# Autodesk Inventor assembly: hintererAufbau
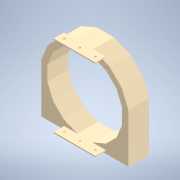
[picture p0: Inventor's stored thumbnail of the model, 180x180]
Saved by Autodesk Inventor 2020.3 (Build 243373010, 373A)
## iProperties
Created: 2021-02-11
Part Number: hintererAufbau
Document SubType Name: Assembly
Designer: Stefan
Author: Stefan
## Documents named in this file (9)
- D:\Stefan\Schule\HTL\Diplomarbeit\git\Inventor\hintererAufbau\hintererAufbau.iam
- D:\Stefan\Schule\HTL\Diplomarbeit\git\Inventor\hintererAufbau\Hauptplatte.ipt
- D:\Stefan\Schule\HTL\Diplomarbeit\git\Inventor\hintererAufbau\InnenUnten.ipt
- D:\Stefan\Schule\HTL\Diplomarbeit\git\Inventor\hintererAufbau\aussenOben.ipt
- D:\Stefan\Schule\HTL\Diplomarbeit\git\Inventor\hintererAufbau\PlatteInnenEineSeite.ipt
- D:\Stefan\Schule\HTL\Diplomarbeit\git\Inventor\hintererAufbau\PlatteInnenzweiSeiten.ipt
- D:\Stefan\Schule\HTL\Diplomarbeit\git\Inventor\hintererAufbau\PlatteAussenEineSeite.ipt
- D:\Stefan\Schule\HTL\Diplomarbeit\git\Inventor\hintererAufbau\PlatteAussenZweiSeiten.ipt
- D:\Stefan\Schule\HTL\Diplomarbeit\git\Inventor\hintererAufbau\PlatteAußenGross.ipt
## Components (27 placed, 8 different names)
1. Hauptplatte:1 — Passend:1, Passend:3, Passend:5, Passend:6, Passend:9, Fluchtend:7, Passend:36, Passend:37, Fluchtend:14, Fluchtend:15, Fluchtend:16, Passend:46, Passend:47, Fluchtend:17, Passend:48, Passend:49, Passend:52, Fluchtend:20
2. Hauptplatte:2 — Passend:2, Passend:4, Fluchtend:1, Passend:7, Fluchtend:2, Passend:8, Fluchtend:3, Passend:11, Passend:12, Passend:13, Passend:14, Passend:15, Passend:16, Passend:17, Passend:18, Fluchtend:4, Passend:19, Fluchtend:5, Passend:20, Passend:21, Fluchtend:6, Passend:22, Passend:23, Passend:24, Passend:25, Fluchtend:8, Passend:26, Passend:27, Fluchtend:9, Passend:28, Passend:29, Fluchtend:10, Passend:30, Passend:31, Passend:32, Fluchtend:11, Passend:33, Fluchtend:12, Passend:34, Passend:35, Fluchtend:13, Passend:38, Passend:39, Passend:40, Passend:41, Passend:42, Passend:43, Passend:44, Passend:45, Fluchtend:18, Passend:50, Passend:51, Fluchtend:19, Passend:53
3. InnenUnten:1 — Passend:1, Passend:2, Passend:3, Passend:4, Fluchtend:1, Passend:5, Passend:10
4. aussenOben:1 — Passend:6, Passend:7, Fluchtend:2, Passend:8
5. PlatteAussenEineSeite:1 — Passend:39, Passend:40
6. PlatteAussenEineSeite:2 — Passend:41, Passend:42
7. PlatteAussenEineSeite:3 — Passend:45, Fluchtend:16, Passend:46
8. PlatteAussenEineSeite:4 — Passend:43, Fluchtend:15, Passend:44
9. PlatteAussenZweiSeiten:1 — Passend:47, Fluchtend:17, Passend:48, Passend:54
10. PlatteAussenZweiSeiten:2 — Passend:49, Fluchtend:18, Passend:50
11. PlatteAußenGross:1 — Passend:53, Passend:54, Fluchtend:20
12. PlatteAußenGross:2 — Passend:51, Passend:52, Fluchtend:19
13. PlatteInnenEineSeite:1 — Passend:9, Fluchtend:3, Passend:10
14. PlatteInnenEineSeite:2 — Passend:14, Passend:16
15. PlatteInnenEineSeite:3 — Passend:13, Passend:15
16. PlatteInnenEineSeite:4 — Passend:11, Passend:12
17. PlatteInnenEineSeite:5 — Passend:17, Passend:18, Fluchtend:4
18. PlatteInnenEineSeite:6 — Passend:21, Fluchtend:6, Passend:22
19. PlatteInnenEineSeite:7 — Passend:23, Fluchtend:7, Passend:24
20. PlatteInnenEineSeite:8 — Passend:27, Fluchtend:9, Passend:28
21. PlatteInnenEineSeite:9 — Passend:31, Passend:32, Fluchtend:11
22. PlatteInnenEineSeite:10 — Passend:35, Passend:36, Fluchtend:13
23. PlatteInnenEineSeite:19 — Passend:33, Fluchtend:12, Passend:34
24. PlatteInnenEineSeite:20 — Passend:29, Fluchtend:10, Passend:30
25. PlatteInnenEineSeite:21 — Passend:25, Fluchtend:8, Passend:26
26. PlatteInnenEineSeite:23 — Passend:19, Fluchtend:5, Passend:20
27. PlatteInnenzweiSeiten:1 — Passend:37, Fluchtend:14, Passend:38
## Relationships (74: Mate 54, Flush 20)
- Passend:1 [Mate]: Hauptplatte:1 ↔ InnenUnten:1
- Passend:2 [Mate]: Hauptplatte:2 ↔ InnenUnten:1
- Passend:3 [Mate]: Hauptplatte:1 ↔ InnenUnten:1
- Passend:4 [Mate]: Hauptplatte:2 ↔ InnenUnten:1
- Fluchtend:1 [Flush]: Hauptplatte:2 ↔ InnenUnten:1
- Passend:5 [Mate]: Hauptplatte:1 ↔ InnenUnten:1
- Passend:6 [Mate]: Hauptplatte:1 ↔ aussenOben:1
- Passend:7 [Mate]: Hauptplatte:2 ↔ aussenOben:1
- Fluchtend:2 [Flush]: Hauptplatte:2 ↔ aussenOben:1
- Passend:8 [Mate]: Hauptplatte:2 ↔ aussenOben:1
- Passend:9 [Mate]: Hauptplatte:1 ↔ PlatteInnenEineSeite:1
- Fluchtend:3 [Flush]: Hauptplatte:2 ↔ PlatteInnenEineSeite:1
- Passend:10 [Mate]: InnenUnten:1 ↔ PlatteInnenEineSeite:1
- Passend:11 [Mate]: Hauptplatte:2 ↔ PlatteInnenEineSeite:4
- Passend:12 [Mate]: Hauptplatte:2 ↔ PlatteInnenEineSeite:4
- Passend:13 [Mate]: Hauptplatte:2 ↔ PlatteInnenEineSeite:3
- Passend:14 [Mate]: Hauptplatte:2 ↔ PlatteInnenEineSeite:2
- Passend:15 [Mate]: Hauptplatte:2 ↔ PlatteInnenEineSeite:3
- Passend:16 [Mate]: Hauptplatte:2 ↔ PlatteInnenEineSeite:2
- Passend:17 [Mate]: Hauptplatte:2 ↔ PlatteInnenEineSeite:5
- Passend:18 [Mate]: Hauptplatte:2 ↔ PlatteInnenEineSeite:5
- Fluchtend:4 [Flush]: Hauptplatte:2 ↔ PlatteInnenEineSeite:5
- Passend:19 [Mate]: Hauptplatte:2 ↔ PlatteInnenEineSeite:23
- Fluchtend:5 [Flush]: Hauptplatte:2 ↔ PlatteInnenEineSeite:23
- Passend:20 [Mate]: Hauptplatte:2 ↔ PlatteInnenEineSeite:23
- Passend:21 [Mate]: Hauptplatte:2 ↔ PlatteInnenEineSeite:6
- Fluchtend:6 [Flush]: Hauptplatte:2 ↔ PlatteInnenEineSeite:6
- Passend:22 [Mate]: Hauptplatte:2 ↔ PlatteInnenEineSeite:6
- Passend:23 [Mate]: Hauptplatte:2 ↔ PlatteInnenEineSeite:7
- Fluchtend:7 [Flush]: Hauptplatte:1 ↔ PlatteInnenEineSeite:7
- Passend:24 [Mate]: Hauptplatte:2 ↔ PlatteInnenEineSeite:7
- Passend:25 [Mate]: Hauptplatte:2 ↔ PlatteInnenEineSeite:21
- Fluchtend:8 [Flush]: Hauptplatte:2 ↔ PlatteInnenEineSeite:21
- Passend:26 [Mate]: Hauptplatte:2 ↔ PlatteInnenEineSeite:21
- Passend:27 [Mate]: Hauptplatte:2 ↔ PlatteInnenEineSeite:8
- Fluchtend:9 [Flush]: Hauptplatte:2 ↔ PlatteInnenEineSeite:8
- Passend:28 [Mate]: Hauptplatte:2 ↔ PlatteInnenEineSeite:8
- Passend:29 [Mate]: Hauptplatte:2 ↔ PlatteInnenEineSeite:20
- Fluchtend:10 [Flush]: Hauptplatte:2 ↔ PlatteInnenEineSeite:20
- Passend:30 [Mate]: Hauptplatte:2 ↔ PlatteInnenEineSeite:20
- Passend:31 [Mate]: Hauptplatte:2 ↔ PlatteInnenEineSeite:9
- Passend:32 [Mate]: Hauptplatte:2 ↔ PlatteInnenEineSeite:9
- Fluchtend:11 [Flush]: Hauptplatte:2 ↔ PlatteInnenEineSeite:9
- Passend:33 [Mate]: Hauptplatte:2 ↔ PlatteInnenEineSeite:19
- Fluchtend:12 [Flush]: Hauptplatte:2 ↔ PlatteInnenEineSeite:19
- Passend:34 [Mate]: Hauptplatte:2 ↔ PlatteInnenEineSeite:19
- Passend:35 [Mate]: Hauptplatte:2 ↔ PlatteInnenEineSeite:10
- Passend:36 [Mate]: Hauptplatte:1 ↔ PlatteInnenEineSeite:10
- Fluchtend:13 [Flush]: Hauptplatte:2 ↔ PlatteInnenEineSeite:10
- Passend:37 [Mate]: Hauptplatte:1 ↔ PlatteInnenzweiSeiten:1
- Fluchtend:14 [Flush]: Hauptplatte:1 ↔ PlatteInnenzweiSeiten:1
- Passend:38 [Mate]: Hauptplatte:2 ↔ PlatteInnenzweiSeiten:1
- Passend:39 [Mate]: Hauptplatte:2 ↔ PlatteAussenEineSeite:1
- Passend:40 [Mate]: Hauptplatte:2 ↔ PlatteAussenEineSeite:1
- Passend:41 [Mate]: Hauptplatte:2 ↔ PlatteAussenEineSeite:2
- Passend:42 [Mate]: Hauptplatte:2 ↔ PlatteAussenEineSeite:2
- Passend:43 [Mate]: Hauptplatte:2 ↔ PlatteAussenEineSeite:4
- Fluchtend:15 [Flush]: Hauptplatte:1 ↔ PlatteAussenEineSeite:4
- Passend:44 [Mate]: Hauptplatte:2 ↔ PlatteAussenEineSeite:4
- Passend:45 [Mate]: Hauptplatte:2 ↔ PlatteAussenEineSeite:3
- Fluchtend:16 [Flush]: Hauptplatte:1 ↔ PlatteAussenEineSeite:3
- Passend:46 [Mate]: Hauptplatte:1 ↔ PlatteAussenEineSeite:3
- Passend:47 [Mate]: Hauptplatte:1 ↔ PlatteAussenZweiSeiten:1
- Fluchtend:17 [Flush]: Hauptplatte:1 ↔ PlatteAussenZweiSeiten:1
- Passend:48 [Mate]: Hauptplatte:1 ↔ PlatteAussenZweiSeiten:1
- Passend:49 [Mate]: Hauptplatte:1 ↔ PlatteAussenZweiSeiten:2
- Fluchtend:18 [Flush]: Hauptplatte:2 ↔ PlatteAussenZweiSeiten:2
- Passend:50 [Mate]: Hauptplatte:2 ↔ PlatteAussenZweiSeiten:2
- Passend:51 [Mate]: Hauptplatte:2 ↔ PlatteAußenGross:2
- Passend:52 [Mate]: Hauptplatte:1 ↔ PlatteAußenGross:2
- Fluchtend:19 [Flush]: Hauptplatte:2 ↔ PlatteAußenGross:2
- Passend:53 [Mate]: Hauptplatte:2 ↔ PlatteAußenGross:1
- Passend:54 [Mate]: PlatteAussenZweiSeiten:1 ↔ PlatteAußenGross:1
- Fluchtend:20 [Flush]: Hauptplatte:1 ↔ PlatteAußenGross:1
